# Autodesk Inventor assembly: Conjunto
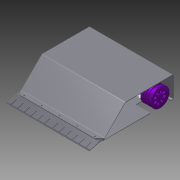
[picture p0: Inventor's stored thumbnail of the model, 180x180]
Saved by Autodesk Inventor 2014 (Build 180170000, 170)
## iProperties
Created: 2014-01-26
Part Number: Conjunto
Document SubType Name: Assembly
Designer: VICTOR
Mass: 1323.68 g
Surface Area: 2356.91 cm^2
Volume: 266.801 cm^3
Density: 4.96132 g/cm^3
Project: ROBOT SUMO
Description: CONJUNTO
Author: Sanjo
Revision Number: 1
## Documents named in this file (7)
- C:\Users\Rubén\Desktop\Kassius\Planos\Conjunto.iam
- C:\Users\Rubén\Desktop\Kassius\Planos\Piezas\Chasis.ipt
- C:\Users\Rubén\Desktop\Kassius\Planos\Piezas\Sub.Rueda.iam
- C:\Users\Rubén\Desktop\Kassius\Planos\Piezas\Cuña.ipt
- C:\Users\Rubén\Desktop\Kassius\Planos\Piezas\Cubierta.ipt
- C:\Users\Rubén\Desktop\Kassius\Planos\Piezas\Servo.ipt
- C:\Users\Rubén\Desktop\Kassius\Planos\Piezas\Leva.ipt
## Components (9 placed, 6 different names)
1. Chasis:1 — Coincidencia:1, Coincidencia:2, Ángulo:1, Ángulo:2, Coincidencia:4, Coincidencia:5, Nivelación:1, Coincidencia:14, Nivelación:2, Coincidencia:15, Nivelación:3, Nivelación:5, Nivelación:6, Coincidencia:17, Coincidencia:18, Coincidencia:19, Coincidencia:20, Coincidencia:21
2. Sub.Rueda:1 [sub-assembly] — Coincidencia:1, Ángulo:1, Coincidencia:3, Coincidencia:4
3. Sub.Rueda:2 [sub-assembly] — Coincidencia:2, Ángulo:2, Coincidencia:3, Coincidencia:5, Nivelación:1
4. Cuña:1 — Coincidencia:14, Nivelación:2, Coincidencia:15
5. Cubierta:1 — Nivelación:3, Nivelación:5, Nivelación:6
6. Servo:1 — Coincidencia:16, Coincidencia:17, Coincidencia:18, Coincidencia:21, Coincidencia:24, Coincidencia:25
7. Servo:2 — Coincidencia:16, Coincidencia:19, Coincidencia:20, Coincidencia:22, Coincidencia:23
8. Leva:1 — Coincidencia:22, Coincidencia:23
9. Leva:2 — Coincidencia:24, Coincidencia:25
## Relationships (24: Mate 17, Flush 5, Angle 2)
- Coincidencia:1 [Mate]: Chasis:1 ↔ Sub.Rueda:1
- Coincidencia:2 [Mate]: Chasis:1 ↔ Sub.Rueda:2
- Ángulo:1 [Angle] (180 deg): Chasis:1 ↔ Sub.Rueda:1
- Ángulo:2 [Angle] (180 deg): Chasis:1 ↔ Sub.Rueda:2
- Coincidencia:3 [Mate]: Sub.Rueda:1 ↔ Sub.Rueda:2
- Coincidencia:4 [Mate] (-5 mm): Chasis:1 ↔ Sub.Rueda:1
- Coincidencia:5 [Mate] (-5 mm): Chasis:1 ↔ Sub.Rueda:2
- Nivelación:1 [Flush] (9 mm): Chasis:1 ↔ Sub.Rueda:2
- Coincidencia:14 [Mate]: Chasis:1 ↔ Cuña:1
- Nivelación:2 [Flush]: Chasis:1 ↔ Cuña:1
- Coincidencia:15 [Mate] (-13 mm): Chasis:1 ↔ Cuña:1
- Nivelación:3 [Flush]: Chasis:1 ↔ Cubierta:1
- Nivelación:5 [Flush]: Chasis:1 ↔ Cubierta:1
- Nivelación:6 [Flush]: Chasis:1 ↔ Cubierta:1
- Coincidencia:16 [Mate]: Servo:1 ↔ Servo:2
- Coincidencia:17 [Mate]: Chasis:1 ↔ Servo:1
- Coincidencia:18 [Mate]: Chasis:1 ↔ Servo:1
- Coincidencia:19 [Mate]: Chasis:1 ↔ Servo:2
- Coincidencia:20 [Mate]: Chasis:1 ↔ Servo:2
- Coincidencia:21 [Mate] (30 mm): Chasis:1 ↔ Servo:1
- Coincidencia:22 [Mate]: Servo:2 ↔ Leva:1
- Coincidencia:23 [Mate]: Servo:2 ↔ Leva:1
- Coincidencia:24 [Mate]: Servo:1 ↔ Leva:2
- Coincidencia:25 [Mate]: Servo:1 ↔ Leva:2
